# Autodesk Inventor assembly: outer_mirrored
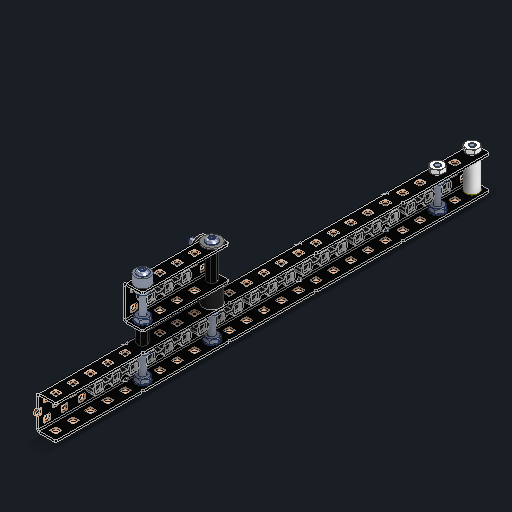
[picture p0: Inventor's stored thumbnail of the model, 512x512]
Saved by Autodesk Inventor 2024 (Build 280153000, 153)
## iProperties
Created: 2024-03-01
Part Number: outer_mirrored
Document SubType Name: Assembly
Designer: Averey Ku
Author: Averey Ku
## Documents named in this file (24)
- D:\vex_robotics\hardware\cad\smolbot\chassis\mirrored_parts\outer_mirrored.iam
- D:\vex_robotics\hardware\cad\smolbot\chassis\mirrored_parts\Alu C 1x2x1x25_mirrored.ipt
- D:\vex_robotics\hardware\cad\smolbot\chassis\mirrored_parts\Bearing Flat Low Profile_mirrored.ipt
- D:\vex_robotics\hardware\cad\smolbot\chassis\mirrored_parts\.375 OD Aluminum Spacer 0.875_mirrored.ipt
- D:\vex_robotics\hardware\cad\smolbot\chassis\mirrored_parts\Nut Keps_mirrored.ipt
- D:\vex_robotics\hardware\cad\VEX-CAD-Inventor-1.41\Structure\Hardware\Screw Steel - Star\SScrew Star Smooth 1.250.ipt
- D:\vex_robotics\hardware\cad\VEX-CAD-Inventor-1.41\Structure\Hardware\Screw Steel - Star.ipt
- D:\vex_robotics\hardware\cad\VEX-CAD-Inventor-1.41\Structure\Hardware\Nut Nylon\Nut Nylon - White.ipt
- D:\vex_robotics\hardware\cad\VEX-CAD-Inventor-1.41\Structure\Hardware\Nut Nylon.ipt
- D:\vex_robotics\hardware\cad\smolbot\chassis\mirrored_parts\Alu C 1x2x1x5_mirrored.ipt
- D:\vex_robotics\hardware\cad\VEX-CAD-Inventor-1.41\Motion\Spacers\Spacer Nylon .500 OD\NSpacer Black .500 OD x .500.ipt
- D:\vex_robotics\hardware\cad\VEX-CAD-Inventor-1.41\Motion\Spacers\Spacer Nylon .500 OD.ipt
- D:\vex_robotics\hardware\cad\VEX-CAD-Inventor-1.41\Structure\Hardware\Screw Steel - Star\SScrew Star Smooth 1.750.ipt
- D:\vex_robotics\hardware\cad\VEX-CAD-Inventor-1.41\Structure\Standoff\Standoff .875.ipt
- D:\vex_robotics\hardware\cad\VEX-CAD-Inventor-1.41\Structure\Standoff.ipt
- D:\vex_robotics\hardware\cad\VEX-CAD-Inventor-1.41\Structure\Standoff\Standoff .50.ipt
- D:\vex_robotics\hardware\cad\VEX-CAD-Inventor-1.41\Structure\Hardware\Screw Shoulder Robosource\SScrew Shoulder Smooth .290 x .09.ipt
- D:\vex_robotics\hardware\cad\VEX-CAD-Inventor-1.41\Structure\Hardware\Screw Shoulder Robosource.ipt
- D:\vex_robotics\hardware\cad\VEX-CAD-Inventor-1.41\Motion\Spacers\Washer Teflon\TWasher .500 OD x .04000.ipt
- D:\vex_robotics\hardware\cad\VEX-CAD-Inventor-1.41\Motion\Spacers\Washer Teflon.ipt
- D:\vex_robotics\hardware\cad\VEX-CAD-Inventor-1.41\Structure\Hardware\Screw Steel - Star\SScrew Star Smooth .375.ipt
- D:\vex_robotics\hardware\cad\smolbot\chassis\mirrored_parts\DWasher .500 OD x .062500_mirrored.ipt
- D:\vex_robotics\hardware\cad\smolbot\chassis\mirrored_parts\Shaft Collar No Screw_mirrored.ipt
- D:\vex_robotics\hardware\cad\VEX-CAD-Inventor-1.41\Structure\Hardware\Screw Steel - Star\SScrew Star Smooth 1.500.ipt
## Components (34 placed, 17 different names)
1. Alu C 1x2x1x25_mirrored:1 — Mate:1, Insert:1, Mate:2, Insert:2, Mate:3, Insert:3, Mate:4, Insert:4, Mate:7, Insert:7, Mate:6, Insert:6, Mate:5, Insert:5, Insert:8, Insert:10, Insert:9, Insert:11, Insert:12, Insert:13, Insert:14, Insert:37, Insert:36, Insert:21, Insert:20, Insert:38, Insert:40, Insert:44, Insert:43
2. Bearing Flat Low Profile_mirrored:1 — Mate:1, Insert:1
3. Bearing Flat Low Profile_mirrored:2 — Mate:2, Insert:2
4. Bearing Flat Low Profile_mirrored:3 — Mate:3, Insert:3
5. Bearing Flat Low Profile_mirrored:4 — Mate:4, Insert:4
6. Bearing Flat Low Profile_mirrored:5 — Mate:7, Insert:7
7. Bearing Flat Low Profile_mirrored:6 — Mate:6, Insert:6
8. Bearing Flat Low Profile_mirrored:7 — Mate:5, Insert:5
9. .375 OD Aluminum Spacer 0.875_mirrored:1 — Insert:8
10. Nut Keps_mirrored:1 — Insert:10
11. Nut Keps_mirrored:2 — Insert:9
12. SScrew Star Smooth 1.250:1 — Insert:11
13. Nut Nylon - White:1 — Insert:12
14. SScrew Star Smooth 1.250:2 — Insert:13
15. Nut Nylon - White:2 — Insert:14
16. Nut Keps_mirrored:3 — Insert:37
17. Nut Keps_mirrored:4 — Insert:36
18. Nut Keps_mirrored:5 — Insert:21
19. Nut Keps_mirrored:6 — Insert:20
20. Bearing Flat Low Profile_mirrored:8 — Mate:9, Insert:34
21. Alu C 1x2x1x5_mirrored:1 — Mate:9, Insert:34, Mate:10, Insert:42, Insert:55, Mate:11, Insert:46, Insert:48, Insert:50, Insert:51, Insert:52, Angle:1, Insert:53
22. NSpacer Black .500 OD x .500:1 — Mate:10, Insert:38
23. SScrew Star Smooth 1.750:3 — Insert:40
24. Standoff .875:1 — Insert:42
25. Standoff .50:2 — Insert:55, Mate:11, Insert:44
26. SScrew Star Smooth 1.250:4 — Insert:43
27. Nut Keps_mirrored:7 — Insert:46
28. SScrew Shoulder Smooth .290 x .09:1 — Insert:49
29. TWasher .500 OD x .04000:1 — Insert:49, Insert:48
30. SScrew Star Smooth .375:5 — Insert:50
31. DWasher .500 OD x .062500_mirrored:1 — Insert:51
32. Nut Keps_mirrored:8 — Insert:52
33. Shaft Collar No Screw_mirrored:1 — Angle:1, Insert:53, Insert:54
34. SScrew Star Smooth 1.500:6 — Insert:54
## Relationships (44: Insert 33, Mate 10, Angle 1)
- Mate:1: Alu C 1x2x1x25_mirrored:1 ↔ Bearing Flat Low Profile_mirrored:1
- Insert:1: Alu C 1x2x1x25_mirrored:1 ↔ Bearing Flat Low Profile_mirrored:1
- Mate:2: Alu C 1x2x1x25_mirrored:1 ↔ Bearing Flat Low Profile_mirrored:2
- Insert:2: Alu C 1x2x1x25_mirrored:1 ↔ Bearing Flat Low Profile_mirrored:2
- Mate:3: Alu C 1x2x1x25_mirrored:1 ↔ Bearing Flat Low Profile_mirrored:3
- Insert:3: Alu C 1x2x1x25_mirrored:1 ↔ Bearing Flat Low Profile_mirrored:3
- Mate:4: Alu C 1x2x1x25_mirrored:1 ↔ Bearing Flat Low Profile_mirrored:4
- Insert:4: Alu C 1x2x1x25_mirrored:1 ↔ Bearing Flat Low Profile_mirrored:4
- Mate:7: Alu C 1x2x1x25_mirrored:1 ↔ Bearing Flat Low Profile_mirrored:5
- Insert:7: Alu C 1x2x1x25_mirrored:1 ↔ Bearing Flat Low Profile_mirrored:5
- Mate:6: Alu C 1x2x1x25_mirrored:1 ↔ Bearing Flat Low Profile_mirrored:6
- Insert:6: Alu C 1x2x1x25_mirrored:1 ↔ Bearing Flat Low Profile_mirrored:6
- Mate:5: Alu C 1x2x1x25_mirrored:1 ↔ Bearing Flat Low Profile_mirrored:7
- Insert:5: Alu C 1x2x1x25_mirrored:1 ↔ Bearing Flat Low Profile_mirrored:7
- Insert:8: Alu C 1x2x1x25_mirrored:1 ↔ .375 OD Aluminum Spacer 0.875_mirrored:1
- Insert:10: Alu C 1x2x1x25_mirrored:1 ↔ Nut Keps_mirrored:1
- Insert:9: Alu C 1x2x1x25_mirrored:1 ↔ Nut Keps_mirrored:2
- Insert:11 (1.5875 mm): Alu C 1x2x1x25_mirrored:1 ↔ SScrew Star Smooth 1.250:1
- Insert:12 (1.5875 mm): Alu C 1x2x1x25_mirrored:1 ↔ Nut Nylon - White:1
- Insert:13 (1.5875 mm): Alu C 1x2x1x25_mirrored:1 ↔ SScrew Star Smooth 1.250:2
- Insert:14 (1.5875 mm): Alu C 1x2x1x25_mirrored:1 ↔ Nut Nylon - White:2
- Insert:37: Alu C 1x2x1x25_mirrored:1 ↔ Nut Keps_mirrored:3
- Insert:36: Alu C 1x2x1x25_mirrored:1 ↔ Nut Keps_mirrored:4
- Insert:21: Alu C 1x2x1x25_mirrored:1 ↔ Nut Keps_mirrored:5
- Insert:20: Alu C 1x2x1x25_mirrored:1 ↔ Nut Keps_mirrored:6
- Mate:9: Bearing Flat Low Profile_mirrored:8 ↔ Alu C 1x2x1x5_mirrored:1
- Insert:34: Bearing Flat Low Profile_mirrored:8 ↔ Alu C 1x2x1x5_mirrored:1
- Mate:10: Alu C 1x2x1x5_mirrored:1 ↔ NSpacer Black .500 OD x .500:1
- Insert:38: Alu C 1x2x1x25_mirrored:1 ↔ NSpacer Black .500 OD x .500:1
- Insert:40: Alu C 1x2x1x25_mirrored:1 ↔ SScrew Star Smooth 1.750:3
- Insert:42: Alu C 1x2x1x5_mirrored:1 ↔ Standoff .875:1
- Insert:55: Alu C 1x2x1x5_mirrored:1 ↔ Standoff .50:2
- Mate:11: Alu C 1x2x1x5_mirrored:1 ↔ Standoff .50:2
- Insert:44: Alu C 1x2x1x25_mirrored:1 ↔ Standoff .50:2
- Insert:43: Alu C 1x2x1x25_mirrored:1 ↔ SScrew Star Smooth 1.250:4
- Insert:46: Alu C 1x2x1x5_mirrored:1 ↔ Nut Keps_mirrored:7
- Insert:49: SScrew Shoulder Smooth .290 x .09:1 ↔ TWasher .500 OD x .04000:1
- Insert:48: Alu C 1x2x1x5_mirrored:1 ↔ TWasher .500 OD x .04000:1
- Insert:50: Alu C 1x2x1x5_mirrored:1 ↔ SScrew Star Smooth .375:5
- Insert:51: Alu C 1x2x1x5_mirrored:1 ↔ DWasher .500 OD x .062500_mirrored:1
- Insert:52: Alu C 1x2x1x5_mirrored:1 ↔ Nut Keps_mirrored:8
- Angle:1 (0 deg): Alu C 1x2x1x5_mirrored:1 ↔ Shaft Collar No Screw_mirrored:1
- Insert:53: Alu C 1x2x1x5_mirrored:1 ↔ Shaft Collar No Screw_mirrored:1
- Insert:54: Shaft Collar No Screw_mirrored:1 ↔ SScrew Star Smooth 1.500:6
